# Autodesk Inventor assembly: Stewart-Body-KST-DS215
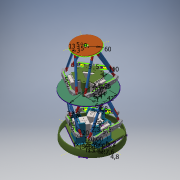
[picture p0: Inventor's stored thumbnail of the model, 180x180]
Saved by Autodesk Inventor 2018.2 (Build 222227000, 227)
## iProperties
Created: 2018-02-24
Part Number: Stewart-Body-KST-DS215
Material: Generisch
Document SubType Name: Assembly
Designer: JochenAlt
Author: JochenAlt
## Documents named in this file (8)
- D:\Projects\Donna\CAD\KST DS215MG\Donna-KST-DS215.iam
- D:\Projects\Donna\CAD\KST DS215MG\Stewart-Base-KST-DS215.iam
- D:\Projects\Donna\CAD\KST DS215MG\Servo-Arm-20mm-Enhanced-Ball-Joint.iam
- D:\Projects\Donna\CAD\KST DS215MG\Body-Rod-KST215MG.iam
- D:\Projects\Donna\CAD\KST DS215MG\Stewart-Body-KST215MG.iam
- D:\Projects\Donna\CAD\KST DS215MG\Servo-Arm-Head-20mm-Ball-Joint.iam
- D:\Projects\Donna\CAD\KST DS215MG\Stewart-Head.iam
- D:\Projects\Donna\CAD\KST DS215MG\Head-Rod-KST215MG.iam
## Components (27 placed, 6 different names)
1. Stewart-Body:1 [sub-assembly] — Passend:55, Passend:57, Passend:60, Passend:62, Passend:64, Passend:65, Passend:66, Passend:67, Passend:68, Passend:69, Passend:70, Passend:71
2. Servo-Arm-20mm-Enhanced-Ball-Joint:1 [sub-assembly] — Passend:17, Passend:64, Passend:70
3. Servo-Arm-20mm-Enhanced-Ball-Joint:2 [sub-assembly] — Passend:16, Passend:65, Passend:68
4. Servo-Arm-20mm-Enhanced-Ball-Joint:3 [sub-assembly] — Passend:15, Passend:60, Passend:66
5. Servo-Arm-20mm-Enhanced-Ball-Joint:4 [sub-assembly] — Passend:13, Passend:62, Passend:71
6. Servo-Arm-20mm-Enhanced-Ball-Joint:5 [sub-assembly] — Passend:18, Passend:55, Passend:69
7. Servo-Arm-20mm-Enhanced-Ball-Joint:6 [sub-assembly] — Passend:14, Passend:57, Passend:67
8. BodyRod-KST215MG:1 [sub-assembly] — Passend:15, Passend:21
9. BodyRod-KST215MG:2 [sub-assembly] — Passend:13, Passend:22
10. BodyRod-KST215MG:3 [sub-assembly] — Passend:14, Passend:23
11. BodyRod-KST215MG:4 [sub-assembly] — Passend:18, Passend:24
12. BodyRod-KST215MG:5 [sub-assembly] — Passend:17, Passend:19
13. BodyRod-KST215MG:6 [sub-assembly] — Passend:16, Passend:20
14. Stewart-Body-KST215MG:1 [sub-assembly] — Passend:19, Passend:20, Passend:21, Passend:22, Passend:23, Passend:24, Passend:49, Passend:50, Passend:51, Passend:52, Passend:53, Passend:54, Passend:72, Passend:73, Passend:74, Passend:75, Passend:76, Passend:77
15. Servo-Arm-Head-20mm-Ball-Joint:1 [sub-assembly] — Passend:39, Passend:49, Passend:73
16. Servo-Arm-Head-20mm-Ball-Joint:2 [sub-assembly] — Passend:40, Passend:50, Passend:72
17. Servo-Arm-Head-20mm-Ball-Joint:3 [sub-assembly] — Passend:42, Passend:54, Passend:76
18. Servo-Arm-Head-20mm-Ball-Joint:4 [sub-assembly] — Passend:41, Passend:53, Passend:77
19. Servo-Arm-Head-20mm-Ball-Joint:5 [sub-assembly] — Passend:37, Passend:52, Passend:74
20. Servo-Arm-Head-20mm-Ball-Joint:6 [sub-assembly] — Passend:38, Passend:51, Passend:75
21. Stewart-Head:1 [sub-assembly] — Passend:43, Passend:44, Passend:45, Passend:46, Passend:47, Passend:48
22. BodyRod-KST215MG:7 [sub-assembly] — Passend:39, Passend:43
23. BodyRod-KST215MG:8 [sub-assembly] — Passend:40, Passend:44
24. BodyRod-KST215MG:9 [sub-assembly] — Passend:41, Passend:47
25. BodyRod-KST215MG:10 [sub-assembly] — Passend:42, Passend:48
26. BodyRod-KST215MG:11 [sub-assembly] — Passend:38, Passend:46
27. BodyRod-KST215MG:12 [sub-assembly] — Passend:37, Passend:45
## Relationships (48: Mate 48)
- Passend:13 [Mate]: Servo-Arm-20mm-Enhanced-Ball-Joint:4 ↔ BodyRod-KST215MG:2
- Passend:14 [Mate]: Servo-Arm-20mm-Enhanced-Ball-Joint:6 ↔ BodyRod-KST215MG:3
- Passend:15 [Mate]: Servo-Arm-20mm-Enhanced-Ball-Joint:3 ↔ BodyRod-KST215MG:1
- Passend:16 [Mate]: Servo-Arm-20mm-Enhanced-Ball-Joint:2 ↔ BodyRod-KST215MG:6
- Passend:17 [Mate]: Servo-Arm-20mm-Enhanced-Ball-Joint:1 ↔ BodyRod-KST215MG:5
- Passend:18 [Mate]: Servo-Arm-20mm-Enhanced-Ball-Joint:5 ↔ BodyRod-KST215MG:4
- Passend:19 [Mate]: BodyRod-KST215MG:5 ↔ Stewart-Body-KST215MG:1
- Passend:20 [Mate]: BodyRod-KST215MG:6 ↔ Stewart-Body-KST215MG:1
- Passend:21 [Mate]: BodyRod-KST215MG:1 ↔ Stewart-Body-KST215MG:1
- Passend:22 [Mate]: BodyRod-KST215MG:2 ↔ Stewart-Body-KST215MG:1
- Passend:23 [Mate]: BodyRod-KST215MG:3 ↔ Stewart-Body-KST215MG:1
- Passend:24 [Mate]: BodyRod-KST215MG:4 ↔ Stewart-Body-KST215MG:1
- Passend:37 [Mate]: Servo-Arm-Head-20mm-Ball-Joint:5 ↔ BodyRod-KST215MG:12
- Passend:38 [Mate]: Servo-Arm-Head-20mm-Ball-Joint:6 ↔ BodyRod-KST215MG:11
- Passend:39 [Mate]: Servo-Arm-Head-20mm-Ball-Joint:1 ↔ BodyRod-KST215MG:7
- Passend:40 [Mate]: Servo-Arm-Head-20mm-Ball-Joint:2 ↔ BodyRod-KST215MG:8
- Passend:41 [Mate]: Servo-Arm-Head-20mm-Ball-Joint:4 ↔ BodyRod-KST215MG:9
- Passend:42 [Mate]: Servo-Arm-Head-20mm-Ball-Joint:3 ↔ BodyRod-KST215MG:10
- Passend:43 [Mate]: Stewart-Head:1 ↔ BodyRod-KST215MG:7
- Passend:44 [Mate]: Stewart-Head:1 ↔ BodyRod-KST215MG:8
- Passend:45 [Mate]: Stewart-Head:1 ↔ BodyRod-KST215MG:12
- Passend:46 [Mate]: Stewart-Head:1 ↔ BodyRod-KST215MG:11
- Passend:47 [Mate]: Stewart-Head:1 ↔ BodyRod-KST215MG:9
- Passend:48 [Mate]: Stewart-Head:1 ↔ BodyRod-KST215MG:10
- Passend:49 [Mate]: Stewart-Body-KST215MG:1 ↔ Servo-Arm-Head-20mm-Ball-Joint:1
- Passend:50 [Mate]: Stewart-Body-KST215MG:1 ↔ Servo-Arm-Head-20mm-Ball-Joint:2
- Passend:51 [Mate]: Stewart-Body-KST215MG:1 ↔ Servo-Arm-Head-20mm-Ball-Joint:6
- Passend:52 [Mate]: Stewart-Body-KST215MG:1 ↔ Servo-Arm-Head-20mm-Ball-Joint:5
- Passend:53 [Mate]: Stewart-Body-KST215MG:1 ↔ Servo-Arm-Head-20mm-Ball-Joint:4
- Passend:54 [Mate]: Stewart-Body-KST215MG:1 ↔ Servo-Arm-Head-20mm-Ball-Joint:3
- Passend:55 [Mate]: Stewart-Body:1 ↔ Servo-Arm-20mm-Enhanced-Ball-Joint:5
- Passend:57 [Mate]: Stewart-Body:1 ↔ Servo-Arm-20mm-Enhanced-Ball-Joint:6
- Passend:60 [Mate]: Stewart-Body:1 ↔ Servo-Arm-20mm-Enhanced-Ball-Joint:3
- Passend:62 [Mate]: Stewart-Body:1 ↔ Servo-Arm-20mm-Enhanced-Ball-Joint:4
- Passend:64 [Mate]: Stewart-Body:1 ↔ Servo-Arm-20mm-Enhanced-Ball-Joint:1
- Passend:65 [Mate]: Stewart-Body:1 ↔ Servo-Arm-20mm-Enhanced-Ball-Joint:2
- Passend:66 [Mate]: Stewart-Body:1 ↔ Servo-Arm-20mm-Enhanced-Ball-Joint:3
- Passend:67 [Mate]: Stewart-Body:1 ↔ Servo-Arm-20mm-Enhanced-Ball-Joint:6
- Passend:68 [Mate]: Stewart-Body:1 ↔ Servo-Arm-20mm-Enhanced-Ball-Joint:2
- Passend:69 [Mate]: Stewart-Body:1 ↔ Servo-Arm-20mm-Enhanced-Ball-Joint:5
- Passend:70 [Mate]: Stewart-Body:1 ↔ Servo-Arm-20mm-Enhanced-Ball-Joint:1
- Passend:71 [Mate]: Stewart-Body:1 ↔ Servo-Arm-20mm-Enhanced-Ball-Joint:4
- Passend:72 [Mate]: Stewart-Body-KST215MG:1 ↔ Servo-Arm-Head-20mm-Ball-Joint:2
- Passend:73 [Mate]: Stewart-Body-KST215MG:1 ↔ Servo-Arm-Head-20mm-Ball-Joint:1
- Passend:74 [Mate]: Stewart-Body-KST215MG:1 ↔ Servo-Arm-Head-20mm-Ball-Joint:5
- Passend:75 [Mate]: Stewart-Body-KST215MG:1 ↔ Servo-Arm-Head-20mm-Ball-Joint:6
- Passend:76 [Mate]: Stewart-Body-KST215MG:1 ↔ Servo-Arm-Head-20mm-Ball-Joint:3
- Passend:77 [Mate]: Stewart-Body-KST215MG:1 ↔ Servo-Arm-Head-20mm-Ball-Joint:4
